# Autodesk Inventor assembly: Mechanism
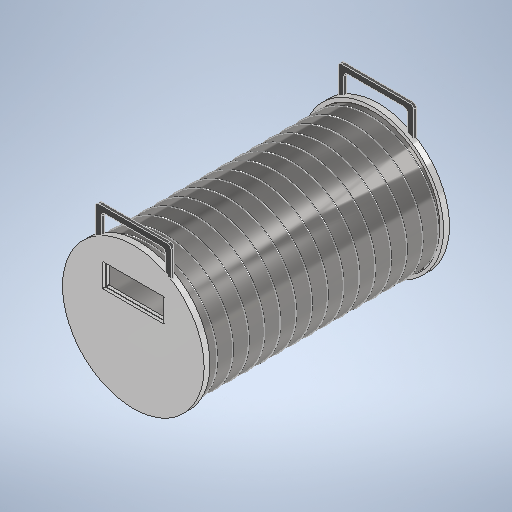
[picture p0: Inventor's stored thumbnail of the model, 512x512]
Saved by Autodesk Inventor 2025.2 (Build 292293000, 293)
## iProperties
Created: 2025-06-02
Part Number: Mechanism
Document SubType Name: Assembly
Designer: dylan
Author: dylan
## Documents named in this file (9)
- C:\Users\gasla\Downloads\Mechanism.iam
- C:\Users\gasla\Downloads\Base Plate.ipt
- C:\Users\gasla\Downloads\Top opening.ipt
- C:\Users\gasla\Downloads\Flap.ipt
- C:\Users\gasla\Downloads\Spring.ipt
- C:\Users\gasla\Downloads\AC25 CAD Mockup\shell.ipt
- C:\Users\gasla\Downloads\Flap_Bottom.ipt
- C:\Users\gasla\Downloads\handlebar.ipt
- C:\Users\gasla\Downloads\handlebar_MIR.ipt
## Components (8 placed, 8 different names)
1. Base Plate:1 — Mate:2, Mate:3, Mate:9, Mate:10, Mate:16, Symmetry:1
2. Spring:1 — Mate:2, Mate:3
3. shell:1 — Mate:9, Mate:10, Mate:11, Mate:12
4. Top opening:1 — Mate:11, Mate:12, Mate:14, Mate:15, Mate:16, Mate:17, Mate:18, Mate:19, Flush:1, Flush:2, Flush:3, Symmetry:1
5. Flap:2 — Mate:14, Mate:15
6. Flap_Bottom:1 — Mate:17, Mate:18, Mate:19
7. handlebar:1 — Flush:1, Flush:2, Flush:3
8. handlebar_MIR:1
## Relationships (16: Mate 12, Flush 3, Symmetry 1)
- Mate:2: Base Plate:1 ↔ Spring:1
- Mate:3: Base Plate:1 ↔ Spring:1
- Mate:9: Base Plate:1 ↔ shell:1
- Mate:10: Base Plate:1 ↔ shell:1
- Mate:11: shell:1 ↔ Top opening:1
- Mate:12: shell:1 ↔ Top opening:1
- Mate:14: Top opening:1 ↔ Flap:2
- Mate:15: Top opening:1 ↔ Flap:2
- Mate:16: Base Plate:1 ↔ Top opening:1
- Mate:17: Top opening:1 ↔ Flap_Bottom:1
- Mate:18: Top opening:1 ↔ Flap_Bottom:1
- Mate:19: Top opening:1 ↔ Flap_Bottom:1
- Flush:1: Top opening:1 ↔ handlebar:1
- Flush:2: Top opening:1 ↔ handlebar:1
- Flush:3: Top opening:1 ↔ handlebar:1
- Symmetry:1: Base Plate:1 ↔ Top opening:1
